# Autodesk Inventor assembly: モータ部分
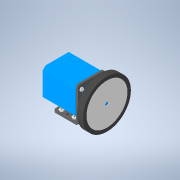
[picture p0: Inventor's stored thumbnail of the model, 180x180]
Saved by Autodesk Inventor 2020 (Build 240168000, 168)
## iProperties
Created: 2020-06-21
Part Number: モータ部分
Document SubType Name: Assembly
Designer: bsat3
Author: bsat3
## Documents named in this file (7)
- C:\Users\haya\Documents\Lecture\ロボット設計製作論４\2020\monotaro\IRC\モータ部分.iam
- C:\Users\haya\Documents\Lecture\ロボット設計製作論４\2020\monotaro\IRC\ステッピングモータ.ipt
- C:\Users\haya\Documents\Lecture\ロボット設計製作論４\2020\monotaro\IRC\ブラケット.ipt
- C:\Users\haya\Documents\Lecture\ロボット設計製作論４\2020\monotaro\IRC\wheel.ipt
- C:\Users\haya\Documents\Lecture\ロボット設計製作論４\2020\monotaro\IRC\tire.ipt
- C:\Users\haya\Documents\Lecture\ロボット設計製作論４\2020\monotaro\IRC\BOB-M3-2-3W.ipt
- C:\Users\haya\Documents\Lecture\ロボット設計製作論４\2020\monotaro\IRC\CSPPN-ST-M3-6_203.ipt
## Components (12 placed, 6 different names)
1. ステッピングモータ:2 — メイト:3, 挿入:2, 挿入:3
2. ブラケット:1 — メイト:3, 挿入:2, 挿入:5, 挿入:6, 挿入:7, 挿入:8, 挿入:9, 挿入:10, 挿入:11, 挿入:12
3. wheel:1 — 挿入:3, 挿入:4
4. tire:1 — 挿入:4
5. BOB-M3-2-3W:1 — 挿入:5
6. BOB-M3-2-3W:2 — 挿入:6
7. BOB-M3-2-3W:3 — 挿入:8
8. BOB-M3-2-3W:4 — 挿入:7
9. CSPPN-ST-M3-6_203:1 — 挿入:9
10. CSPPN-ST-M3-6_203:2 — 挿入:10
11. CSPPN-ST-M3-6_203:3 — 挿入:12
12. CSPPN-ST-M3-6_203:4 — 挿入:11
## Relationships (12: Insert 11, Mate 1)
- メイト:3 [Mate]: ステッピングモータ:2 ↔ ブラケット:1
- 挿入:2 [Insert]: ステッピングモータ:2 ↔ ブラケット:1
- 挿入:3 [Insert] (-1 mm): ステッピングモータ:2 ↔ wheel:1
- 挿入:4 [Insert]: wheel:1 ↔ tire:1
- 挿入:5 [Insert]: ブラケット:1 ↔ BOB-M3-2-3W:1
- 挿入:6 [Insert]: ブラケット:1 ↔ BOB-M3-2-3W:2
- 挿入:7 [Insert]: ブラケット:1 ↔ BOB-M3-2-3W:4
- 挿入:8 [Insert]: ブラケット:1 ↔ BOB-M3-2-3W:3
- 挿入:9 [Insert]: ブラケット:1 ↔ CSPPN-ST-M3-6_203:1
- 挿入:10 [Insert]: ブラケット:1 ↔ CSPPN-ST-M3-6_203:2
- 挿入:11 [Insert]: ブラケット:1 ↔ CSPPN-ST-M3-6_203:4
- 挿入:12 [Insert]: ブラケット:1 ↔ CSPPN-ST-M3-6_203:3
